# Autodesk Inventor assembly: UBG-Sensoreinheit
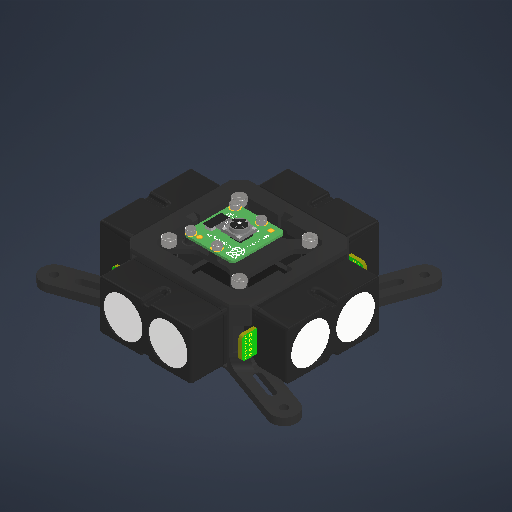
[picture p0: Inventor's stored thumbnail of the model, 512x512]
Saved by Autodesk Inventor 2025.2 (Build 292293000, 293)
## iProperties
Created: 2025-03-28
Part Number: UBG-Sensoreinheit
Document SubType Name: Assembly
Designer: Faabs
Author: Faabs
## Documents named in this file (10)
- C:\Users\Faabs\Desktop\TeamFaabs-CAD v2023\UBG\Sensoreinheit\UBG-Sensoreinheit.iam
- C:\Users\Faabs\Desktop\TeamFaabs-CAD v2023\OBG\Grundkoerper_Lidar\Grundkoerper_Lidar\Grundkoerper_Lidar.ipt
- C:\Users\Faabs\Desktop\TeamFaabs-CAD v2023\UBG\LidarGarmin Lite v4\UBG-LidarGarmin.iam
- C:\Users\Faabs\Desktop\TeamFaabs-CAD v2023\Verbindungselemente\Abstandsbolzen_Kamera.ipt
- C:\Users\Faabs\Desktop\TeamFaabs-CAD v2023\Platinen\I2C-Platine\I2C-Platine\I2C-Platine.ipt
- C:\Users\Faabs\Desktop\TeamFaabs-CAD v2023\UBG\Sensoreinheit\Cam V2\Cam V2\Cam V2.ipt
- C:\Users\Faabs\Desktop\TeamFaabs-CAD v2023\UBG\Sensoreinheit\Kamerahalterung\Kamerahalterung\Kamerahalterung.ipt
- C:\Users\Faabs\Desktop\TeamFaabs-CAD v2023\Verbindungselemente\DIN 912\DIN 912 - M2 x 0,4 x 6 x 5.ipt
- C:\Users\Faabs\Desktop\TeamFaabs-CAD v2023\Verbindungselemente\DIN 912\DIN 912 - M3 x 0,5 x 6 x 4,75.ipt
- C:\Users\Faabs\Desktop\TeamFaabs-CAD v2023\Verbindungselemente\DIN 7991\DIN 7991 - M3x8.ipt
## Components (24 placed, 9 different names)
1. Grundkoerper_Lidar:1 — Fluchtend:1, Fluchtend:2, Passend:1, Passend:3, Passend:4, Passend:5, Passend:6, Passend:7, Einfügen:13, Einfügen:14, Einfügen:15, Einfügen:16
2. Abstandsbolzen_Kamera:1 — Einfügen:2, Passend:10
3. Abstandsbolzen_Kamera:2 — Einfügen:1, Passend:9
4. Abstandsbolzen_Kamera:3 — Einfügen:3, Passend:8
5. Abstandsbolzen_Kamera:4 — Einfügen:4
6. I2C-Platine:1 — Passend:5, Passend:6, Passend:7, Einfügen:1, Einfügen:2, Einfügen:3, Einfügen:4
7. Cam V2:1 — Passend:11, Passend:12, Passend:13, Einfügen:5, Einfügen:6, Einfügen:7, Einfügen:8
8. Kamerahalterung:1 — Passend:8, Passend:9, Passend:10, Passend:11, Passend:12, Passend:13, Einfügen:9, Einfügen:10, Einfügen:11, Einfügen:12
9. DIN 7991 M3x8:1 — Einfügen:16
10. DIN 7991 M3x8:2 — Einfügen:13
11. DIN 7991 M3x8:3 — Einfügen:14
12. DIN 7991 M3x8:4 — Einfügen:15
13. DIN 912 - ersetzt durch DIN EN ISO 4762 M2 x 6:1 — Einfügen:8
14. DIN 912 - ersetzt durch DIN EN ISO 4762 M2 x 6:2 — Einfügen:7
15. DIN 912 - ersetzt durch DIN EN ISO 4762 M2 x 6:3 — Einfügen:6
16. DIN 912 - ersetzt durch DIN EN ISO 4762 M2 x 6:4 — Einfügen:5
17. DIN 912 - ersetzt durch DIN EN ISO 4762 M3 x 6:1 — Einfügen:9
18. DIN 912 - ersetzt durch DIN EN ISO 4762 M3 x 6:2 — Einfügen:10
19. DIN 912 - ersetzt durch DIN EN ISO 4762 M3 x 6:3 — Einfügen:12
20. DIN 912 - ersetzt durch DIN EN ISO 4762 M3 x 6:4 — Einfügen:11
21. UBG-LidarGarmin:1 [sub-assembly] — Fluchtend:3, Passend:3, Passend:4
22. UBG-LidarGarmin:2 [sub-assembly]
23. UBG-LidarGarmin:3 [sub-assembly]
24. UBG-LidarGarmin:4 [sub-assembly]
## Component patterns: (4 elements, first: UBG-LidarGarmin:1)
## Relationships (31: Insert 16, Mate 12, Flush 3)
- Fluchtend:1 [Flush]: Grundkoerper_Lidar:1
- Fluchtend:2 [Flush]: Grundkoerper_Lidar:1
- Passend:1 [Mate]: Grundkoerper_Lidar:1
- Fluchtend:3 [Flush]: UBG-LidarGarmin:1
- Passend:3 [Mate]: Grundkoerper_Lidar:1 ↔ UBG-LidarGarmin:1
- Passend:4 [Mate]: Grundkoerper_Lidar:1 ↔ UBG-LidarGarmin:1
- Passend:5 [Mate]: Grundkoerper_Lidar:1 ↔ I2C-Platine:1
- Passend:6 [Mate]: Grundkoerper_Lidar:1 ↔ I2C-Platine:1
- Passend:7 [Mate]: Grundkoerper_Lidar:1 ↔ I2C-Platine:1
- Einfügen:1 [Insert]: Abstandsbolzen_Kamera:2 ↔ I2C-Platine:1
- Einfügen:2 [Insert]: Abstandsbolzen_Kamera:1 ↔ I2C-Platine:1
- Einfügen:3 [Insert]: Abstandsbolzen_Kamera:3 ↔ I2C-Platine:1
- Einfügen:4 [Insert]: Abstandsbolzen_Kamera:4 ↔ I2C-Platine:1
- Passend:8 [Mate]: Abstandsbolzen_Kamera:3 ↔ Kamerahalterung:1
- Passend:9 [Mate]: Abstandsbolzen_Kamera:2 ↔ Kamerahalterung:1
- Passend:10 [Mate]: Abstandsbolzen_Kamera:1 ↔ Kamerahalterung:1
- Passend:11 [Mate]: Cam V2:1 ↔ Kamerahalterung:1
- Passend:12 [Mate]: Cam V2:1 ↔ Kamerahalterung:1
- Passend:13 [Mate]: Cam V2:1 ↔ Kamerahalterung:1
- Einfügen:5 [Insert]: Cam V2:1 ↔ DIN 912 - ersetzt durch DIN EN ISO 4762 M2 x 6:4
- Einfügen:6 [Insert]: Cam V2:1 ↔ DIN 912 - ersetzt durch DIN EN ISO 4762 M2 x 6:3
- Einfügen:7 [Insert]: Cam V2:1 ↔ DIN 912 - ersetzt durch DIN EN ISO 4762 M2 x 6:2
- Einfügen:8 [Insert]: Cam V2:1 ↔ DIN 912 - ersetzt durch DIN EN ISO 4762 M2 x 6:1
- Einfügen:9 [Insert]: Kamerahalterung:1 ↔ DIN 912 - ersetzt durch DIN EN ISO 4762 M3 x 6:1
- Einfügen:10 [Insert]: Kamerahalterung:1 ↔ DIN 912 - ersetzt durch DIN EN ISO 4762 M3 x 6:2
- Einfügen:11 [Insert]: Kamerahalterung:1 ↔ DIN 912 - ersetzt durch DIN EN ISO 4762 M3 x 6:4
- Einfügen:12 [Insert]: Kamerahalterung:1 ↔ DIN 912 - ersetzt durch DIN EN ISO 4762 M3 x 6:3
- Einfügen:13 [Insert]: Grundkoerper_Lidar:1 ↔ DIN 7991 M3x8:2
- Einfügen:14 [Insert]: Grundkoerper_Lidar:1 ↔ DIN 7991 M3x8:3
- Einfügen:15 [Insert]: Grundkoerper_Lidar:1 ↔ DIN 7991 M3x8:4
- Einfügen:16 [Insert]: Grundkoerper_Lidar:1 ↔ DIN 7991 M3x8:1
